# Autodesk Inventor assembly: Tamale Assembly Plate Assembly V3
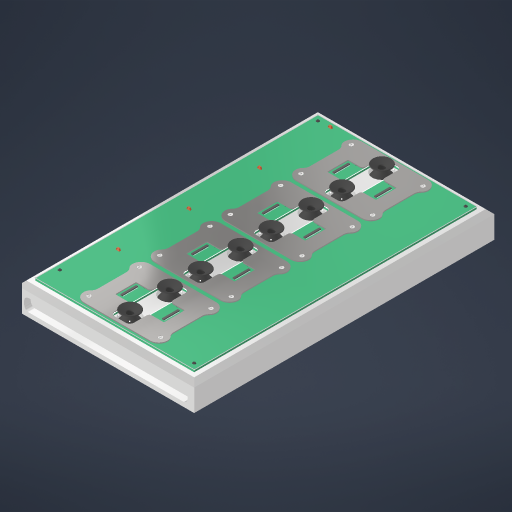
[picture p0: Inventor's stored thumbnail of the model, 512x512]
Saved by Autodesk Inventor 2024 (Build 280153000, 153)
## iProperties
Created: 2022-03-23
Part Number: Tamale Assembly Plate Assembly V3
Document SubType Name: Assembly
Designer: Caleb
Author: Caleb
## Documents named in this file (9)
- C:\Users\cfangmeier3\Desktop\nebraska-silicon-lab\Hardware\ETL\Module Assembly\Tamale Assembly Plate V3\Tamale Assembly Plate Assembly V3.iam
- C:\Users\cfangmeier3\Desktop\nebraska-silicon-lab\Hardware\ETL\Module Assembly\Tamale Assembly Plate V3\Tamale Assembly Plate V3.ipt
- C:\Users\cfangmeier3\Desktop\nebraska-silicon-lab\Hardware\ETL\Module Assembly\Tamale Assembly Plate V3\5427A624_Vacuum Cup.ipt
- C:\Users\cfangmeier3\Desktop\nebraska-silicon-lab\Hardware\ETL\Module Assembly\Tamale Assembly Plate V3\spacer.ipt
- C:\Users\cfangmeier3\Desktop\nebraska-silicon-lab\Hardware\ETL\Module Assembly\Tamale Assembly Plate V3\91771A054_Passivated 18-8 Stainless Steel Phillips Flat Head Screw.ipt
- C:\Users\cfangmeier3\Desktop\nebraska-silicon-lab\Hardware\ETL\Module Assembly\Tamale Assembly Plate V3\90910A443_BUTTON HEAD TORX SCREWS.ipt
- C:\Users\cfangmeier3\Desktop\nebraska-silicon-lab\Hardware\ETL\Module Assembly\Tamale Assembly Plate V3\etl_assembly_plate_pcb_v3.ipt
- C:\Users\cfangmeier3\Desktop\nebraska-silicon-lab\Hardware\ETL\modules\throughput mockups\Throughput Mockup Assembly.iam
- C:\Users\cfangmeier3\Desktop\nebraska-silicon-lab\Hardware\ETL\Module Assembly\Tamale Assembly Plate V3\Module PCB Edge Clip.ipt
## Components (36 placed, 8 different names)
1. Tamale Assembly Plate V3:1 — Angle:1, Insert:1, Insert:14, Insert:15, Angle:3, Angle:4
2. 90910A443_BUTTON HEAD TORX SCREWS:1
3. 90910A443_BUTTON HEAD TORX SCREWS:2
4. 90910A443_BUTTON HEAD TORX SCREWS:3
5. 90910A443_BUTTON HEAD TORX SCREWS:4
6. etl_assembly_plate_pcb_v3:1 — Insert:15, Angle:2
7. Throughput Mockup Assembly:1 [sub-assembly] — Angle:2, Angle:3
8. Module PCB Edge Clip:1 — Angle:4
9. 91771A054_Passivated 18-8 Stainless Steel Phillips Flat Head Screw:2 — Insert:5
10. 91771A054_Passivated 18-8 Stainless Steel Phillips Flat Head Screw:4 — Insert:7
11. spacer:1 — Insert:4, Insert:5, Insert:6, Insert:7
12. 5427A624_Vacuum Cup:1 — Angle:1, Insert:1
13. 5427A624_Vacuum Cup:2 — Insert:14
14. 91771A054_Passivated 18-8 Stainless Steel Phillips Flat Head Screw:1 — Insert:4
15. 91771A054_Passivated 18-8 Stainless Steel Phillips Flat Head Screw:3 — Insert:6
16. 91771A054_Passivated 18-8 Stainless Steel Phillips Flat Head Screw:5
17. 91771A054_Passivated 18-8 Stainless Steel Phillips Flat Head Screw:6
18. spacer:2
19. 5427A624_Vacuum Cup:3
20. 5427A624_Vacuum Cup:4
21. 91771A054_Passivated 18-8 Stainless Steel Phillips Flat Head Screw:7
22. 91771A054_Passivated 18-8 Stainless Steel Phillips Flat Head Screw:8
23. 91771A054_Passivated 18-8 Stainless Steel Phillips Flat Head Screw:9
24. 91771A054_Passivated 18-8 Stainless Steel Phillips Flat Head Screw:10
25. spacer:3
26. 5427A624_Vacuum Cup:5
27. 5427A624_Vacuum Cup:6
28. 91771A054_Passivated 18-8 Stainless Steel Phillips Flat Head Screw:11
29. 91771A054_Passivated 18-8 Stainless Steel Phillips Flat Head Screw:12
30. 91771A054_Passivated 18-8 Stainless Steel Phillips Flat Head Screw:13
31. 91771A054_Passivated 18-8 Stainless Steel Phillips Flat Head Screw:14
32. spacer:4
33. 5427A624_Vacuum Cup:7
34. 5427A624_Vacuum Cup:8
35. 91771A054_Passivated 18-8 Stainless Steel Phillips Flat Head Screw:15
36. 91771A054_Passivated 18-8 Stainless Steel Phillips Flat Head Screw:16
## Component patterns: (4 elements, first: 91771A054_Passivated 18-8 Stainless Steel Phillips Flat Head Screw:2 + 91771A054_Passivated 18-8 Stainless Steel Phillips Flat Head Screw:4 + spacer:1 + 5427A624_Vacuum Cup:1 + 5427A624_Vacuum Cup:2 + 91771A054_Passivated 18-8 Stainless Steel Phillips Flat Head Screw:1 + 91771A054_Passivated 18-8 Stainless Steel Phillips Flat Head Screw:3)
## Relationships (11: Insert 7, Angle 4)
- Angle:1 (0 deg): Tamale Assembly Plate V3:1 ↔ 5427A624_Vacuum Cup:1
- Insert:1: Tamale Assembly Plate V3:1 ↔ 5427A624_Vacuum Cup:1
- Insert:4: spacer:1 ↔ 91771A054_Passivated 18-8 Stainless Steel Phillips Flat Head Screw:1
- Insert:5: 91771A054_Passivated 18-8 Stainless Steel Phillips Flat Head Screw:2 ↔ spacer:1
- Insert:6: spacer:1 ↔ 91771A054_Passivated 18-8 Stainless Steel Phillips Flat Head Screw:3
- Insert:7: 91771A054_Passivated 18-8 Stainless Steel Phillips Flat Head Screw:4 ↔ spacer:1
- Insert:14: Tamale Assembly Plate V3:1 ↔ 5427A624_Vacuum Cup:2
- Insert:15: Tamale Assembly Plate V3:1 ↔ etl_assembly_plate_pcb_v3:1
- Angle:2 (0 deg): etl_assembly_plate_pcb_v3:1 ↔ Throughput Mockup Assembly:1
- Angle:3 (0 deg): Tamale Assembly Plate V3:1 ↔ Throughput Mockup Assembly:1
- Angle:4 (0 deg): Tamale Assembly Plate V3:1 ↔ Module PCB Edge Clip:1
